# Autodesk Inventor assembly: Window_Cabinet
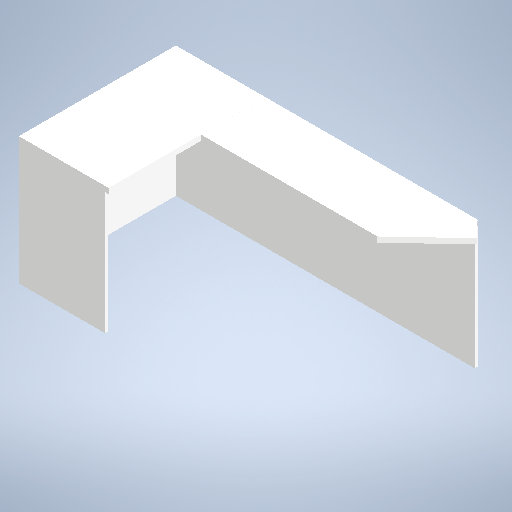
[picture p0: Inventor's stored thumbnail of the model, 512x512]
Saved by Autodesk Inventor 2025 (Build 290162000, 162)
## iProperties
Created: 2023-05-06
Part Number: Window_Cabinet
Document SubType Name: Assembly
Designer: Tom
Author: Tom
## Documents named in this file (6)
- C:\Users\Tom\Documents\Mobility\First_Floor\Window_Cabinet\Window_Cabinet.iam
- C:\Users\Tom\Documents\Mobility\First_Floor\Window_Cabinet\Plywood--0.75_x_34_x_77.25_in.ipt
- C:\Users\Tom\Documents\Mobility\First_Floor\Window_Cabinet\Butcher_Block--1.5_x_25_x_43.75_in.ipt
- C:\Users\Tom\Documents\Mobility\First_Floor\Window_Cabinet\Plywood--0.75_x_34_x_23.25_in.ipt
- C:\Users\Tom\Documents\Mobility\First_Floor\Window_Cabinet\Quartz_Countertop--1.5_x_18_x_63.34829.ipt
- C:\Users\Tom\Documents\Mobility\First_Floor\Window_Cabinet\Plywood--0.75_x_34_x_42.75_in.ipt
## Components (5 placed, 5 different names)
1. Plywood--0.75_x_34_x_77.25_in:1 — Flush:7, Mate:4, Mate:5, Mate:8, Flush:12, Flush:13, Flush:16
2. Plywood--0.75_x_34_x_23.25_in:2 — Flush:14, Flush:15, Mate:9
3. Butcher_Block--1.5_x_25_x_43.75_in:2 — Flush:7, Mate:4, Mate:6
4. Quartz_Countertop--1.5_x_18_x_63.34829:1 — Mate:5, Mate:6, Flush:16
5. Plywood--0.75_x_34_x_42.75_in:1 — Mate:8, Flush:12, Flush:13, Flush:14, Flush:15, Mate:9
## Relationships (11: Flush 6, Mate 5)
- Flush:7: Plywood--0.75_x_34_x_77.25_in:1 ↔ Butcher_Block--1.5_x_25_x_43.75_in:2
- Mate:4: Plywood--0.75_x_34_x_77.25_in:1 ↔ Butcher_Block--1.5_x_25_x_43.75_in:2
- Mate:5: Plywood--0.75_x_34_x_77.25_in:1 ↔ Quartz_Countertop--1.5_x_18_x_63.34829:1
- Mate:6: Butcher_Block--1.5_x_25_x_43.75_in:2 ↔ Quartz_Countertop--1.5_x_18_x_63.34829:1
- Mate:8: Plywood--0.75_x_34_x_77.25_in:1 ↔ Plywood--0.75_x_34_x_42.75_in:1
- Flush:12: Plywood--0.75_x_34_x_77.25_in:1 ↔ Plywood--0.75_x_34_x_42.75_in:1
- Flush:13: Plywood--0.75_x_34_x_77.25_in:1 ↔ Plywood--0.75_x_34_x_42.75_in:1
- Flush:14: Plywood--0.75_x_34_x_23.25_in:2 ↔ Plywood--0.75_x_34_x_42.75_in:1
- Flush:15: Plywood--0.75_x_34_x_23.25_in:2 ↔ Plywood--0.75_x_34_x_42.75_in:1
- Mate:9: Plywood--0.75_x_34_x_23.25_in:2 ↔ Plywood--0.75_x_34_x_42.75_in:1
- Flush:16: Plywood--0.75_x_34_x_77.25_in:1 ↔ Quartz_Countertop--1.5_x_18_x_63.34829:1
